# Autodesk Inventor assembly: CompleteRobotAssembly_NERDS
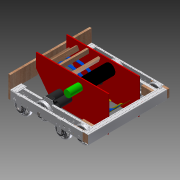
[picture p0: Inventor's stored thumbnail of the model, 180x180]
Saved by Autodesk Inventor 2014 (Build 180170000, 170)
## iProperties
Created: 2016-01-30
Part Number: CompleteRobotAssembly_NERDS
Document SubType Name: Assembly
Designer: bermudezr
Author: bermudezr
## Documents named in this file (3)
- C:\Users\choices.CTE\Documents\Nerds_1726\Models\2015-2016\Assemblies\Robot\Complete.iam
- C:\Users\choices.CTE\Documents\Nerds_1726\Models\2015-2016\Assemblies\Robot\Shooter.iam
- C:\Users\choices.CTE\Documents\Nerds_1726\Models\2015-2016\Assemblies\Robot\Chassis.iam
## Components (2 placed, 2 different names)
1. Shooter:1 [sub-assembly] — Mate:1, Mate:2, Flush:1
2. Chassis:1 [sub-assembly] — Mate:1, Mate:2, Flush:1
## Relationships (3: Mate 2, Flush 1)
- Mate:1: Shooter:1 ↔ Chassis:1
- Mate:2: Shooter:1 ↔ Chassis:1
- Flush:1: Shooter:1 ↔ Chassis:1
